# Autodesk Inventor assembly: button
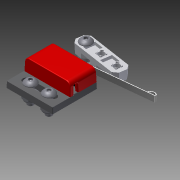
[picture p0: Inventor's stored thumbnail of the model, 180x180]
Saved by Autodesk Inventor 2014 SP1 (Build 180222100, 222)
## iProperties
Created: 2014-04-14
Part Number: button
Document SubType Name: Assembly
Designer: Ryan
Author: Ryan
## Documents named in this file (7)
- C:\Users\Ryan\Desktop\sw\toss up 5th A bot\tower\button.iam
- C:\Users\Ryan\Desktop\sw\lib\Super Sonic Sparks VEX CAD Library\Motors & Sensors\Limit Switch (Sensor).iam
- C:\Users\Ryan\Desktop\sw\lib\Aperture VEX CAD Library\Metal\C Channel\2 x 4.ipt
- C:\Users\Ryan\Desktop\sw\lib\Aperture VEX CAD Library\Hardware\8-32\8-32_.500.ipt
- C:\Users\Ryan\Desktop\sw\lib\Aperture VEX CAD Library\Hardware\8-32\8-32 nylock.ipt
- C:\Users\Ryan\Desktop\sw\lib\Aperture VEX CAD Library\Spacers\thin\SPACER-0320-0125.ipt
- C:\Users\Ryan\Desktop\sw\lib\Aperture VEX CAD Library\Bearing Blocks\Bearing Block.ipt
## Components (10 placed, 6 different names)
1. Limit Switch (Sensor):1 [sub-assembly] — Mate:1, Mate:2, Mate:3, Mate:5, Mate:22
2. 2 x 4:1 — Mate:1, Mate:2, Mate:3, Mate:6, Mate:7, Mate:8, Mate:12, Mate:13, Mate:14, Mate:16, Mate:19, Mate:20, Mate:21
3. 8-32 nylock:1 — Mate:4, Mate:6
4. 8-32_.500:1 — Mate:4, Mate:5, Mate:7, Mate:8
5. SPACER-0320-0125:1 — Mate:10, Mate:11, Mate:12
6. 8-32_.500:3 — Mate:15, Mate:23
7. 8-32 nylock:3 — Mate:16
8. Bearing Block:1 — Mate:10, Mate:11, Mate:13, Mate:14, Mate:15, Mate:23
9. 8-32_.500:4 — Mate:20, Mate:21, Mate:22
10. 8-32 nylock:4 — Mate:19
## Relationships (22: Mate 22)
- Mate:1: Limit Switch (Sensor):1 ↔ 2 x 4:1
- Mate:2 (2.3114 mm): Limit Switch (Sensor):1 ↔ 2 x 4:1
- Mate:3 (-12.7 mm): Limit Switch (Sensor):1 ↔ 2 x 4:1
- Mate:4: 8-32 nylock:1 ↔ 8-32_.500:1
- Mate:5: Limit Switch (Sensor):1 ↔ 8-32_.500:1
- Mate:6: 2 x 4:1 ↔ 8-32 nylock:1
- Mate:7 (2.3114 mm): 2 x 4:1 ↔ 8-32_.500:1
- Mate:8 (2.3114 mm): 2 x 4:1 ↔ 8-32_.500:1
- [Mate]: 8-32_.500:3 ↔ 8-32 nylock:3
- Mate:10: SPACER-0320-0125:1 ↔ Bearing Block:1
- Mate:11: SPACER-0320-0125:1 ↔ Bearing Block:1
- Mate:12: 2 x 4:1 ↔ SPACER-0320-0125:1
- Mate:13 (2.3114 mm): 2 x 4:1 ↔ Bearing Block:1
- Mate:14 (2.3114 mm): 2 x 4:1 ↔ Bearing Block:1
- Mate:15: 8-32_.500:3 ↔ Bearing Block:1
- Mate:16: 2 x 4:1 ↔ 8-32 nylock:3
- [Mate]: 8-32_.500:4 ↔ 8-32 nylock:4
- Mate:19: 2 x 4:1 ↔ 8-32 nylock:4
- Mate:20 (2.3114 mm): 2 x 4:1 ↔ 8-32_.500:4
- Mate:21 (2.3114 mm): 2 x 4:1 ↔ 8-32_.500:4
- Mate:22: Limit Switch (Sensor):1 ↔ 8-32_.500:4
- Mate:23: 8-32_.500:3 ↔ Bearing Block:1
## Named parameters: q = 2.3114 mm, d13_d3 = 0 mm, d21_d3 = 0 mm
